# Autodesk Inventor assembly: GFRP_T2_02
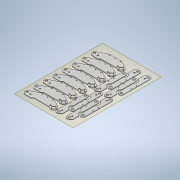
[picture p0: Inventor's stored thumbnail of the model, 180x180]
Saved by Autodesk Inventor 2020 (Build 240168000, 168)
## iProperties
Created: 2021-08-27
Part Number: GFRP_T2_02
Document SubType Name: Assembly
Designer: Masato
Author: Masato
## Documents named in this file (4)
- C:\Users\naoki\Documents\Inventor\CitBrains\git_clone\OpenPlatform167\CAMの確認用\OpenPlatform_ver3_0\cam\GFRP_T2_02.iam
- C:\Users\naoki\Documents\Inventor\CitBrains\git_clone\OpenPlatform167\CAMの確認用\OpenPlatform_ver3_0\cam\Disposable_Board.ipt
- C:\Users\naoki\Documents\Inventor\CitBrains\git_clone\OpenPlatform167\CAMの確認用\OpenPlatform_ver3_0\LowerBody\Link\BackLink_frame.ipt
- C:\Users\naoki\Documents\Inventor\CitBrains\git_clone\OpenPlatform167\CAMの確認用\OpenPlatform_ver3_0\LowerBody\Link\FrontLink_frame.ipt
## Components (17 placed, 3 different names)
1. Disposable_Board:1 — メイト:2, メイト:1, フラッシュ:1, フラッシュ:2, フラッシュ:3, 正接:3, 角度:1, フラッシュ:4, メイト:7, 正接:5
2. FrontLink_frame:1 — メイト:4, フラッシュ:3, 正接:3
3. FrontLink_frame:2
4. FrontLink_frame:3
5. FrontLink_frame:4
6. FrontLink_frame:5
7. FrontLink_frame:6
8. FrontLink_frame:7
9. FrontLink_frame:8
10. BackLink_frame:1 — メイト:5, 角度:1, フラッシュ:4, メイト:6, 正接:4
11. BackLink_frame:2 — メイト:6, メイト:7, 正接:4, 正接:5
12. BackLink_frame:3
13. BackLink_frame:4
14. BackLink_frame:5
15. BackLink_frame:6
16. BackLink_frame:7
17. BackLink_frame:8
## Component patterns: (8 elements, first: FrontLink_frame:1), (4 elements, first: BackLink_frame:1 + BackLink_frame:2)
## Relationships (14: Mate 6, Flush 4, Tangent 3, Angle 1)
- メイト:2 [Mate]: Disposable_Board:1
- メイト:1 [Mate]: Disposable_Board:1
- フラッシュ:1 [Flush]: Disposable_Board:1
- フラッシュ:2 [Flush]: Disposable_Board:1
- メイト:4 [Mate]: FrontLink_frame:1
- フラッシュ:3 [Flush] (2 mm): Disposable_Board:1 ↔ FrontLink_frame:1
- 正接:3 [Tangent] (2 mm): Disposable_Board:1 ↔ FrontLink_frame:1
- メイト:5 [Mate]: BackLink_frame:1
- 角度:1 [Angle] (0 deg): Disposable_Board:1 ↔ BackLink_frame:1
- フラッシュ:4 [Flush] (2.5 mm): Disposable_Board:1 ↔ BackLink_frame:1
- メイト:6 [Mate] (2.5 mm): BackLink_frame:1 ↔ BackLink_frame:2
- メイト:7 [Mate]: Disposable_Board:1 ↔ BackLink_frame:2
- 正接:4 [Tangent] (2.5 mm): BackLink_frame:1 ↔ BackLink_frame:2
- 正接:5 [Tangent] (2 mm): Disposable_Board:1 ↔ BackLink_frame:2
